# Autodesk Inventor assembly: SquareSupport
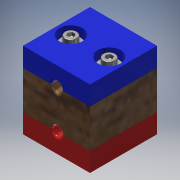
[picture p0: Inventor's stored thumbnail of the model, 180x180]
Saved by Autodesk Inventor 2017 SP1 (Build 210196100, 196)
## iProperties
Created: 2015-12-11
Part Number: SquareSupport
Document SubType Name: Assembly
Designer: steele
Author: steele
## Documents named in this file (6)
- D:\snobotics\CAD-Development\robSteele\HouseProjects\Garage\SquareSupport.iam
- D:\snobotics\CAD-Development\robSteele\HouseProjects\Garage\BottomOfSquareSupport.ipt
- D:\snobotics\CAD-Development\robSteele\HouseProjects\Garage\MiddleOfSquareSupport.ipt
- D:\snobotics\CAD-Development\robSteele\HouseProjects\Garage\TopOfSquareSupport.ipt
- D:\snobotics\CAD-Development\robSteele\HouseProjects\Garage\SquareSupport\Design Accelerator\Bolted Connection2.iam
- D:\snobotics\CAD-Development\robSteele\HouseProjects\Garage\SquareSupport\Design Accelerator\Bolted Connection3.iam
## Components (5 placed, 4 different names)
1. BottomOfSquareSupport:1 — Mate:1, Flush:1, Flush:2
2. MiddleOfSquareSupport:1 — Mate:1, Flush:1, Flush:2, Mate:5, Flush:3, Flush:4
3. TopOfSquareSupport:1 — Mate:5, Flush:3, Flush:4, Mate:6, Mate:7, Mate:8, Mate:9
4. Bolted Connection:1 [sub-assembly] — Mate:6, Mate:7
5. Bolted Connection:2 [sub-assembly] — Mate:8, Mate:9
## Relationships (10: Mate 6, Flush 4)
- Mate:1: BottomOfSquareSupport:1 ↔ MiddleOfSquareSupport:1
- Flush:1: BottomOfSquareSupport:1 ↔ MiddleOfSquareSupport:1
- Flush:2: BottomOfSquareSupport:1 ↔ MiddleOfSquareSupport:1
- Mate:5: MiddleOfSquareSupport:1 ↔ TopOfSquareSupport:1
- Flush:3: MiddleOfSquareSupport:1 ↔ TopOfSquareSupport:1
- Flush:4: MiddleOfSquareSupport:1 ↔ TopOfSquareSupport:1
- Mate:6: TopOfSquareSupport:1 ↔ Bolted Connection:1
- Mate:7: TopOfSquareSupport:1 ↔ Bolted Connection:1
- Mate:8: TopOfSquareSupport:1 ↔ Bolted Connection:2
- Mate:9: TopOfSquareSupport:1 ↔ Bolted Connection:2
## Named parameters: bottomHoleDiam = 9.525 mm, width = 38.1 mm, heightOfBottomHole = 11.1125 mm, deltaBottomToTop = 25.4 mm, heightOfTopHole = 11.1125 mm, topHoleDiam = 9.525 mm, edgeToBoltHole = 7.14375 mm, height = 47.625 mm
